# Autodesk Inventor assembly: Blockhaus
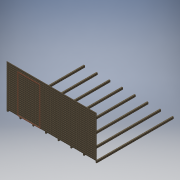
[picture p0: Inventor's stored thumbnail of the model, 180x180]
Saved by Autodesk Inventor 2017 (Build 210142000, 142)
## iProperties
Created: 2017-05-11
Part Number: Blockhaus
Document SubType Name: Assembly
Designer: Fake
Author: Fake
## Documents named in this file (4)
- C:\Users\Fake\Documents\Inventor\Oli_Grundstück\Blockhaus.iam
- C:\Users\Fake\Documents\Inventor\Oli_Grundstück\Bodenbalken.ipt
- C:\Users\Fake\Documents\Inventor\Oli_Grundstück\Brett_vorne.ipt
- C:\Users\Fake\Documents\Inventor\Oli_Grundstück\Rahmen.iam
## Components (33 placed, 3 different names)
1. Rahmen:1 [sub-assembly] — Passend:2, Passend:3
2. Bodenbalken:1 — Passend:1, Fluchtend:2, Passend:3
3. Bodenbalken:2
4. Bodenbalken:3
5. Bodenbalken:4
6. Bodenbalken:5
7. Bodenbalken:6
8. Bodenbalken:7
9. Bodenbalken:8
10. Brett_vorne:1 — Fluchtend:1, Passend:1, Fluchtend:2, Passend:2
11. Brett_vorne:2
12. Brett_vorne:3
13. Brett_vorne:4
14. Brett_vorne:5
15. Brett_vorne:6
16. Brett_vorne:7
17. Brett_vorne:8
18. Brett_vorne:9
19. Brett_vorne:10
20. Brett_vorne:11
21. Brett_vorne:12
22. Brett_vorne:13
23. Brett_vorne:14
24. Brett_vorne:15
25. Brett_vorne:16
26. Brett_vorne:17
27. Brett_vorne:18
28. Brett_vorne:19
29. Brett_vorne:20
30. Brett_vorne:21
31. Brett_vorne:22
32. Brett_vorne:23
33. Brett_vorne:24
## Component patterns: (8 elements, first: Bodenbalken:1), (24 elements, first: Brett_vorne:1)
## Relationships (5: Mate 3, Flush 2)
- Fluchtend:1 [Flush]: Brett_vorne:1
- Passend:1 [Mate]: Bodenbalken:1 ↔ Brett_vorne:1
- Fluchtend:2 [Flush]: Bodenbalken:1 ↔ Brett_vorne:1
- Passend:2 [Mate]: Rahmen:1 ↔ Brett_vorne:1
- Passend:3 [Mate]: Rahmen:1 ↔ Bodenbalken:1
